# Autodesk Inventor assembly: I53
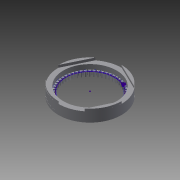
[picture p0: Inventor's stored thumbnail of the model, 180x180]
Saved by Autodesk Inventor 2014 (Build 180170000, 170)
## iProperties
Created: 2013-05-25
Part Number: I53
Document SubType Name: Assembly
Designer: Felix
Author: Felix
## Documents named in this file (4)
- C:\Users\Felix\Desktop\Beep\Hardware\Z132053\I53.iam
- C:\Users\Felix\Desktop\Beep\Hardware\Z132053\Z53.ipt
- C:\Users\Felix\Desktop\Beep\Hardware\Z132053\I53O.ipt
- C:\Users\Felix\Desktop\snap.ipt
## Components (4 placed, 3 different names)
1. Z53:1 — Mate:1, Flush:1
2. I53O:1 — Flush:1, Flush:3
3. snap:1
4. snap:2 — Flush:3, Mate:2
## Relationships (4: Mate 2, Flush 2)
- Mate:1: Z53:1
- Flush:1: Z53:1 ↔ I53O:1
- Flush:3: I53O:1 ↔ snap:2
- Mate:2: snap:2
